# Autodesk Inventor assembly: exhaust header right
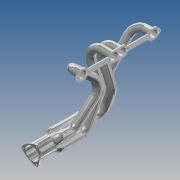
[picture p0: Inventor's stored thumbnail of the model, 180x180]
Saved by Autodesk Inventor 2013 (Build 170138000, 138)
## iProperties
Created: 2013-02-09
Part Number: exhaust header right
Document SubType Name: Assembly
Designer: zhaphod
Author: zhaphod
## Documents named in this file (8)
- C:\drawings\vette\chevy engine\exhaust header right.iam
- C:\drawings\vette\chevy engine\exhaust header plate.ipt
- C:\drawings\vette\chevy engine\exhaust header right pipe 8.ipt
- C:\drawings\vette\chevy engine\exhaust header collector.ipt
- C:\drawings\vette\chevy engine\exhaust header right pipe 7.ipt
- C:\drawings\vette\chevy engine\exhaust header right pipe 5.ipt
- C:\drawings\vette\chevy engine\exhaust header right pipe 3.ipt
- C:\drawings\vette\chevy engine\exhaust header right pipe 1.ipt
## Components (7 placed, 7 different names)
1. exhaust header plate:1 — Mate:1, Flush:1, Mate:2, Mate:3, Mate:4, Flush:2, Flush:3, Flush:4, Mate:9, Flush:5, Flush:6, Flush:7, Flush:8, Flush:9
2. exhaust header right pipe 8:1 — Mate:1, Flush:1
3. exhaust header right pipe 5:1 — Mate:3, Flush:4, Flush:9
4. exhaust header right pipe 3:1 — Mate:2, Flush:3, Flush:8
5. exhaust header right pipe 1:1 — Mate:4, Flush:2, Flush:7, Mate:12
6. exhaust header collector:1 — Mate:10, Mate:11, Mate:12
7. exhaust header right pipe 7:1 — Mate:9, Flush:5, Flush:6, Mate:10, Mate:11
## Relationships (17: Flush 9, Mate 8)
- Mate:1: exhaust header plate:1 ↔ exhaust header right pipe 8:1
- Flush:1: exhaust header plate:1 ↔ exhaust header right pipe 8:1
- Mate:2: exhaust header plate:1 ↔ exhaust header right pipe 3:1
- Mate:3: exhaust header plate:1 ↔ exhaust header right pipe 5:1
- Mate:4: exhaust header plate:1 ↔ exhaust header right pipe 1:1
- Flush:2: exhaust header plate:1 ↔ exhaust header right pipe 1:1
- Flush:3: exhaust header plate:1 ↔ exhaust header right pipe 3:1
- Flush:4: exhaust header plate:1 ↔ exhaust header right pipe 5:1
- Mate:9: exhaust header plate:1 ↔ exhaust header right pipe 7:1
- Flush:5: exhaust header plate:1 ↔ exhaust header right pipe 7:1
- Flush:6: exhaust header plate:1 ↔ exhaust header right pipe 7:1
- Flush:7: exhaust header plate:1 ↔ exhaust header right pipe 1:1
- Flush:8: exhaust header plate:1 ↔ exhaust header right pipe 3:1
- Flush:9: exhaust header plate:1 ↔ exhaust header right pipe 5:1
- Mate:10 (-38.1 mm): exhaust header collector:1 ↔ exhaust header right pipe 7:1
- Mate:11: exhaust header collector:1 ↔ exhaust header right pipe 7:1
- Mate:12: exhaust header right pipe 1:1 ↔ exhaust header collector:1
